# Autodesk Inventor assembly: ASY GBK центральная стенка
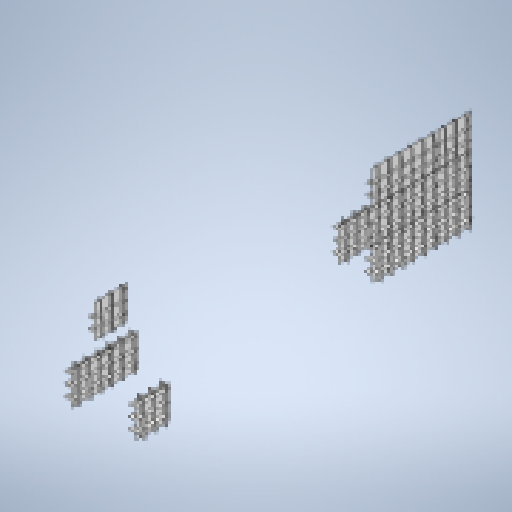
[picture p0: Inventor's stored thumbnail of the model, 512x512]
Saved by Autodesk Inventor 2026 (Build 300175000, 175)
## iProperties
Created: 2026-05-28
Part Number: ASY GBK центральная стенка
Document SubType Name: Assembly
Designer: pokla
Author: pokla
## Documents named in this file (10)
- C:\Users\pokla\Documents\Inventor\GBK-Gubkinskiy\ASY GBK центральная стенка.iam
- C:\Users\pokla\Documents\Inventor\GBK-Gubkinskiy\ASY GBK 3110 central wall shield 1.iam
- C:\Users\pokla\Documents\Inventor\GBK-Gubkinskiy\ASY GBK 3120 central wall shield 2.iam
- C:\Users\pokla\Documents\Inventor\GBK-Gubkinskiy\ASY GBK 3210 central wall shield 3.iam
- C:\Users\pokla\Documents\Inventor\GBK-Gubkinskiy\ASY GBK 3220 central wall shield 4.iam
- C:\Users\pokla\Documents\Inventor\GBK-Gubkinskiy\ASY GBK 3310 central wall shield 5.iam
- C:\Users\pokla\Documents\Inventor\GBK-Gubkinskiy\ASY GBK 3320 central wall shield 8.iam
- C:\Users\pokla\Documents\Inventor\GBK-Gubkinskiy\ASY GBK 3330 central wall shield 9.iam
- C:\Users\pokla\Documents\Inventor\GBK-Gubkinskiy\ASY GBK 3230 central wall shield 6.iam
- C:\Users\pokla\Documents\Inventor\GBK-Gubkinskiy\ASY GBK 3130 central wall shield 3.iam
## Components (9 placed, 9 different names)
1. ASY GBK 3110 central wall shield 1:1 [sub-assembly] — Совмещение:1, Совмещение:3, Жесткий:1, Совмещение:4, Жесткий:2
2. ASY GBK 3120 central wall shield 2:1 [sub-assembly] — Жесткий:1
3. ASY GBK 3210 central wall shield 3:1 [sub-assembly] — Жесткий:2, Жесткий:3, Жесткий:4
4. ASY GBK 3220 central wall shield 4:1 [sub-assembly] — Жесткий:3
5. ASY GBK 3310 central wall shield 5:1 [sub-assembly] — Жесткий:4, Жесткий:5
6. ASY GBK 3320 central wall shield 8:1 [sub-assembly] — Жесткий:5
7. ASY GBK 3330 central wall shield 9:1 [sub-assembly]
8. ASY GBK 3230 central wall shield 6:1 [sub-assembly]
9. ASY GBK 3130 central wall shield 3:1 [sub-assembly]
## Relationships (8: WeldJoint 5, Mate 3)
- Совмещение:1 [Mate]: ASY GBK 3110 central wall shield 1:1
- Совмещение:3 [Mate]: ASY GBK 3110 central wall shield 1:1
- Жесткий:1 [WeldJoint] (1 mm): ASY GBK 3110 central wall shield 1:1 ↔ ASY GBK 3120 central wall shield 2:1
- Совмещение:4 [Mate]: ASY GBK 3110 central wall shield 1:1
- Жесткий:2 [WeldJoint]: ASY GBK 3110 central wall shield 1:1 ↔ ASY GBK 3210 central wall shield 3:1
- Жесткий:3 [WeldJoint] (1 mm): ASY GBK 3210 central wall shield 3:1 ↔ ASY GBK 3220 central wall shield 4:1
- Жесткий:4 [WeldJoint]: ASY GBK 3210 central wall shield 3:1 ↔ ASY GBK 3310 central wall shield 5:1
- Жесткий:5 [WeldJoint] (1 mm): ASY GBK 3310 central wall shield 5:1 ↔ ASY GBK 3320 central wall shield 8:1
